# Autodesk Inventor assembly: main
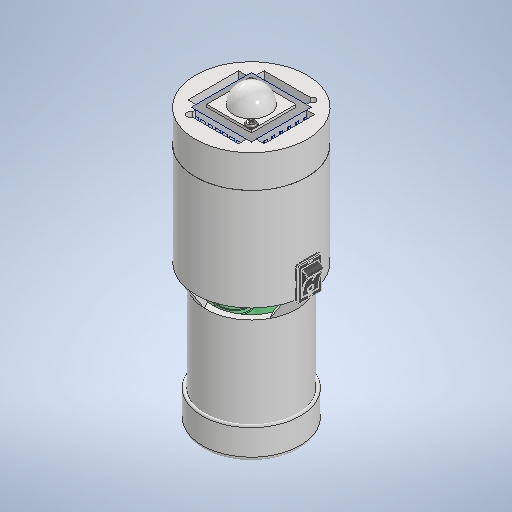
[picture p0: Inventor's stored thumbnail of the model, 512x512]
Saved by Autodesk Inventor 2025 (Build 290162000, 162)
## iProperties
Created: 2025-08-17
Part Number: main
Document SubType Name: Assembly
Designer: gavin
Author: gavin
## Documents named in this file (10)
- D:\Inventor\super flashlight v4\main.iam
- D:\Inventor\super flashlight v4\outercase.ipt
- D:\Inventor\super flashlight v4\super flash light v4 head.ipt
- D:\Inventor\super flashlight v4\super flash light v4.ipt
- D:\Inventor\super flashlight v4\Mini Rocker 4-Pin Switch\Mini Rocker 4-Pin Switch.ipt
- D:\Inventor\super flashlight v4\Sony Murata VTC5A 18650 2600mAh 25A Battery\Sony Murata VTC5A 18650 2600mAh 25A Battery.ipt
- D:\Inventor\super flashlight v4\heatsink.ipt
- D:\Inventor\super flashlight v4\40mm x 40mm x 28mm Fan Assy\40mm x 40mm x 28mm Fan Assy.ipt
- D:\Inventor\super flashlight v4\50w led.ipt
- D:\Inventor\super flashlight v4\AS 1427 - M3 x 6(5) II.ipt
## Components (13 placed, 9 different names)
1. outercase:1 — 剛性:1, 剛性:2, 貼合:1, 貼合:2, 相切:1, 齊平:4, 相切:7, 相切:8, 相切:9
2. super flash light v4 head:1 — 剛性:2, 貼合:3, 齊平:5, 貼合:4, 貼合:5, 貼合:6
3. super flash light v4:1 — 剛性:1
4. Mini Rocker 4-Pin Switch:1 — 貼合:1, 貼合:2, 相切:1
5. Sony Murata VTC5A 18650 2600mAh 25A Battery:1 — 相切:2, 齊平:1, 齊平:2, 相切:5, 齊平:3, 齊平:4, 相切:7
6. Sony Murata VTC5A 18650 2600mAh 25A Battery:2 — 相切:5, 齊平:3, 相切:6, 相切:9
7. Sony Murata VTC5A 18650 2600mAh 25A Battery:3 — 相切:2, 齊平:1, 相切:3, 相切:8
8. Sony Murata VTC5A 18650 2600mAh 25A Battery:4 — 相切:3, 齊平:2, 相切:6
9. heatsink:1 — 貼合:3, 齊平:5, 貼合:4, 貼合:7, 貼合:8, 貼合:9
10. 40mm x 40mm x 28mm Fan Assy:1 — 貼合:5, 貼合:6
11. 50w led:1 — 貼合:7, 貼合:8, 貼合:9, 剛性:3, 剛性:4
12. AS 1427 - M3 x 6(5) II:1 — 剛性:3
13. AS 1427 - M3 x 6(5) II:2 — 剛性:4
## Relationships (26: Mate 9, Tangent 8, Flush 5, WeldJoint 4)
- 剛性:1 [WeldJoint]: outercase:1 ↔ super flash light v4:1
- 剛性:2 [WeldJoint]: outercase:1 ↔ super flash light v4 head:1
- 貼合:1 [Mate]: outercase:1 ↔ Mini Rocker 4-Pin Switch:1
- 貼合:2 [Mate]: outercase:1 ↔ Mini Rocker 4-Pin Switch:1
- 相切:1 [Tangent]: outercase:1 ↔ Mini Rocker 4-Pin Switch:1
- 相切:2 [Tangent]: Sony Murata VTC5A 18650 2600mAh 25A Battery:1 ↔ Sony Murata VTC5A 18650 2600mAh 25A Battery:3
- 齊平:1 [Flush]: Sony Murata VTC5A 18650 2600mAh 25A Battery:1 ↔ Sony Murata VTC5A 18650 2600mAh 25A Battery:3
- 相切:3 [Tangent]: Sony Murata VTC5A 18650 2600mAh 25A Battery:3 ↔ Sony Murata VTC5A 18650 2600mAh 25A Battery:4
- 齊平:2 [Flush]: Sony Murata VTC5A 18650 2600mAh 25A Battery:1 ↔ Sony Murata VTC5A 18650 2600mAh 25A Battery:4
- 相切:5 [Tangent]: Sony Murata VTC5A 18650 2600mAh 25A Battery:1 ↔ Sony Murata VTC5A 18650 2600mAh 25A Battery:2
- 齊平:3 [Flush]: Sony Murata VTC5A 18650 2600mAh 25A Battery:1 ↔ Sony Murata VTC5A 18650 2600mAh 25A Battery:2
- 相切:6 [Tangent]: Sony Murata VTC5A 18650 2600mAh 25A Battery:2 ↔ Sony Murata VTC5A 18650 2600mAh 25A Battery:4
- 齊平:4 [Flush]: outercase:1 ↔ Sony Murata VTC5A 18650 2600mAh 25A Battery:1
- 相切:7 [Tangent]: outercase:1 ↔ Sony Murata VTC5A 18650 2600mAh 25A Battery:1
- 相切:8 [Tangent]: outercase:1 ↔ Sony Murata VTC5A 18650 2600mAh 25A Battery:3
- 相切:9 [Tangent]: outercase:1 ↔ Sony Murata VTC5A 18650 2600mAh 25A Battery:2
- 貼合:3 [Mate]: super flash light v4 head:1 ↔ heatsink:1
- 齊平:5 [Flush]: super flash light v4 head:1 ↔ heatsink:1
- 貼合:4 [Mate]: super flash light v4 head:1 ↔ heatsink:1
- 貼合:5 [Mate] (0.25 mm): super flash light v4 head:1 ↔ 40mm x 40mm x 28mm Fan Assy:1
- 貼合:6 [Mate] (0.25 mm): super flash light v4 head:1 ↔ 40mm x 40mm x 28mm Fan Assy:1
- 貼合:7 [Mate]: heatsink:1 ↔ 50w led:1
- 貼合:8 [Mate]: heatsink:1 ↔ 50w led:1
- 貼合:9 [Mate]: heatsink:1 ↔ 50w led:1
- 剛性:3 [WeldJoint]: 50w led:1 ↔ AS 1427 - M3 x 6(5) II:1
- 剛性:4 [WeldJoint]: 50w led:1 ↔ AS 1427 - M3 x 6(5) II:2
